# Autodesk Inventor assembly: SE Matriz Centelladora DC
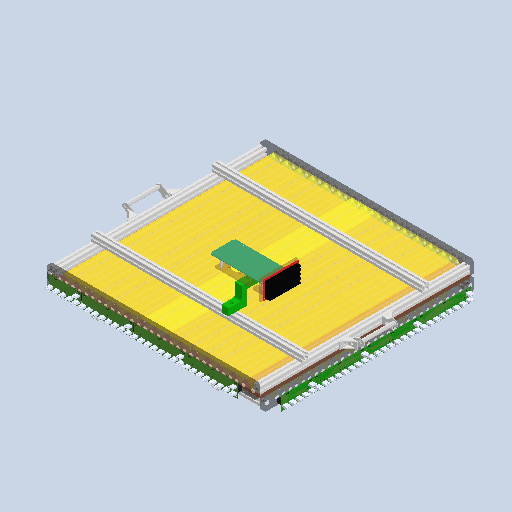
[picture p0: Inventor's stored thumbnail of the model, 512x512]
Saved by Autodesk Inventor 2024.2 (Build 282272000, 272)
## iProperties
Created: 2025-11-07
Part Number: SE Matriz Centelladora DC
Document SubType Name: Assembly
Designer: ja.restrepo1
Author: ja.restrepo1
## Documents named in this file (8)
- I:\MICROMECANICA\ALTAS ENERGIAS\Deteccion de Muones\Detectores centelladores\Partes Detector Centellador\SE Matriz Centelladora DC\SE Matriz Centelladora DC.iam
- I:\MICROMECANICA\ALTAS ENERGIAS\Deteccion de Muones\Detectores centelladores\Partes Detector Centellador\SE Matriz Centelladora DC\Soporte de matriz centelladora.ipt
- I:\MICROMECANICA\ALTAS ENERGIAS\Deteccion de Muones\Detectores centelladores\Partes Detector Centellador\SE Matriz Centelladora DC\SSE Matriz Centelladora 15X14\SSE Matriz centelladora 15X14.iam
- I:\MICROMECANICA\ALTAS ENERGIAS\Deteccion de Muones\Detectores centelladores\Partes Detector Centellador\SE Matriz Centelladora DC\SSE Estructura Centelladoras 20x20 DC\SSE estructura matriz centelladora.iam
- I:\MICROMECANICA\ALTAS ENERGIAS\Deteccion de Muones\Detectores centelladores\Partes Detector Centellador\SE Matriz Centelladora DC\SSE Manija\SSE. Manija.iam
- I:\MICROMECANICA\ALTAS ENERGIAS\Deteccion de Muones\Detectores centelladores\Partes Detector Centellador\SE Tarjetas IC DC\SSE tarjedas de AD DC.iam
- I:\MICROMECANICA\ALTAS ENERGIAS\Deteccion de Muones\Detectores centelladores\Partes Detector Centellador\SE Tarjetas IC DC\SSE SiPM 8CH Org.iam
- I:\MICROMECANICA\ALTAS ENERGIAS\Deteccion de Muones\Detectores centelladores\Partes Detector Centellador\SE Tarjetas IC DC\SSE SiPM 8Ch_2026.iam
## Components (10 placed, 7 different names)
1. Soporte de matriz centelladora:1 — Flush:1, Flush:2, Flush:3, Mate:1, Mate:2, Flush:4, Flush:5, Mate:3, Flush:6, Flush:7, Mate:4, Flush:8, Flush:9, Flush:10, Flush:11
2. SSE Matriz centelladora 15X14:1 [sub-assembly] — Mate:2, Flush:4, Flush:6, Flush:7
3. SSE Matriz centelladora 15X14:2 [sub-assembly] — Flush:5, Mate:3, Mate:4
4. SSE estructura matriz centelladora:1 [sub-assembly] — Flush:8, Flush:9, Flush:10, Mate:5, Flush:12, Mate:6, Flush:13, Mate:7, Angle:1, Flush:15, Mate:8, Angle:2, Mate:9, Flush:16, Mate:10, Mate:11, Flush:17, Flush:18, Mate:12, Mate:13
5. SSE. Manija:1 [sub-assembly] — Mate:5, Flush:11, Flush:12, Flush:14
6. SSE. Manija:2 [sub-assembly] — Mate:6, Flush:13, Flush:14
7. SSE tarjedas de AD DC:1 [sub-assembly] — Mate:7, Angle:1, Flush:15
8. SSE SiPM 8CH Org:1 [sub-assembly] — Mate:10, Mate:11, Flush:17
9. SSE SiPM 8CH Org:2 [sub-assembly] — Mate:8, Angle:2, Mate:9, Flush:16
10. SSE SiPM 8Ch_2026:1 [sub-assembly] — Flush:18, Mate:12, Mate:13
## Relationships (33: Flush 18, Mate 13, Angle 2)
- Flush:1: Soporte de matriz centelladora:1
- Flush:2: Soporte de matriz centelladora:1
- Flush:3: Soporte de matriz centelladora:1
- Mate:1: Soporte de matriz centelladora:1
- Mate:2: Soporte de matriz centelladora:1 ↔ SSE Matriz centelladora 15X14:1
- Flush:4: Soporte de matriz centelladora:1 ↔ SSE Matriz centelladora 15X14:1
- Flush:5: Soporte de matriz centelladora:1 ↔ SSE Matriz centelladora 15X14:2
- Mate:3: Soporte de matriz centelladora:1 ↔ SSE Matriz centelladora 15X14:2
- Flush:6: Soporte de matriz centelladora:1 ↔ SSE Matriz centelladora 15X14:1
- Flush:7: Soporte de matriz centelladora:1 ↔ SSE Matriz centelladora 15X14:1
- Mate:4: Soporte de matriz centelladora:1 ↔ SSE Matriz centelladora 15X14:2
- Flush:8: Soporte de matriz centelladora:1 ↔ SSE estructura matriz centelladora:1
- Flush:9: Soporte de matriz centelladora:1 ↔ SSE estructura matriz centelladora:1
- Flush:10: Soporte de matriz centelladora:1 ↔ SSE estructura matriz centelladora:1
- Mate:5: SSE estructura matriz centelladora:1 ↔ SSE. Manija:1
- Flush:11: Soporte de matriz centelladora:1 ↔ SSE. Manija:1
- Flush:12 (0.5 mm): SSE estructura matriz centelladora:1 ↔ SSE. Manija:1
- Mate:6: SSE estructura matriz centelladora:1 ↔ SSE. Manija:2
- Flush:13 (-0.5 mm): SSE estructura matriz centelladora:1 ↔ SSE. Manija:2
- Flush:14: SSE. Manija:1 ↔ SSE. Manija:2
- Mate:7: SSE estructura matriz centelladora:1 ↔ SSE tarjedas de AD DC:1
- Angle:1 (0 deg): SSE estructura matriz centelladora:1 ↔ SSE tarjedas de AD DC:1
- Flush:15 (-9 mm): SSE estructura matriz centelladora:1 ↔ SSE tarjedas de AD DC:1
- Mate:8 (10 mm): SSE estructura matriz centelladora:1 ↔ SSE SiPM 8CH Org:2
- Angle:2 (0 deg): SSE estructura matriz centelladora:1 ↔ SSE SiPM 8CH Org:2
- Mate:9 (3 mm): SSE estructura matriz centelladora:1 ↔ SSE SiPM 8CH Org:2
- Flush:16: SSE estructura matriz centelladora:1 ↔ SSE SiPM 8CH Org:2
- Mate:10 (10 mm): SSE estructura matriz centelladora:1 ↔ SSE SiPM 8CH Org:1
- Mate:11 (3 mm): SSE estructura matriz centelladora:1 ↔ SSE SiPM 8CH Org:1
- Flush:17: SSE estructura matriz centelladora:1 ↔ SSE SiPM 8CH Org:1
- Flush:18: SSE estructura matriz centelladora:1 ↔ SSE SiPM 8Ch_2026:1
- Mate:12 (10 mm): SSE estructura matriz centelladora:1 ↔ SSE SiPM 8Ch_2026:1
- Mate:13: SSE estructura matriz centelladora:1 ↔ SSE SiPM 8Ch_2026:1
